# Autodesk Inventor assembly: ASY Мешалка
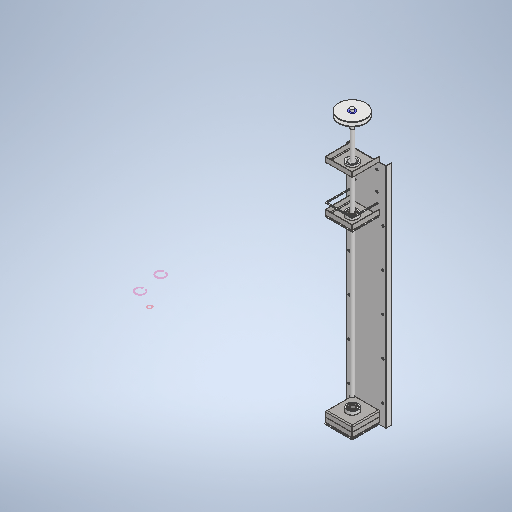
[picture p0: Inventor's stored thumbnail of the model, 512x512]
Saved by Autodesk Inventor 2025 (Build 290162010, 162A)
## iProperties
Created: 2024-04-09
Part Number: ASY Мешалка
Document SubType Name: Assembly
Designer: pokla
Author: pokla
## Documents named in this file (14)
- C:\Users\pokla\Documents\Inventor\Мешалка\ASY Мешалка.iam
- C:\Users\pokla\Documents\Inventor\Мешалка\SKF B7203 BE.ipt
- C:\Users\pokla\Documents\Inventor\Мешалка\Вал.ipt
- C:\Users\pokla\Documents\Inventor\Мешалка\дистанс.втулка.ipt
- C:\Users\pokla\Documents\Inventor\Мешалка\Втулка.ipt
- C:\Users\pokla\Documents\Inventor\Мешалка\CSN 02 9401 - G 17x40x7 - NBR.ipt
- C:\Users\pokla\Documents\Inventor\Мешалка\Шкив 119 мм.ipt
- Шкив 119 мм.ipt
- C:\Users\pokla\Documents\Inventor\Мешалка\Втулка для шкива.ipt
- C:\Users\pokla\Documents\Inventor\Content Center Files\R2024\en-US\ANSI B 27.7M(2)\ANSI B 27.7M - 3AMI-17.ipt
- C:\Users\pokla\Documents\Inventor\Content Center Files\R2024\en-US\ANSI B 27.7M(1)\ANSI B 27.7M - 3BMI-40.ipt
- C:\Users\pokla\Documents\Inventor\Мешалка\ASY Мешалка 2.0.iam
- C:\Users\pokla\Documents\Inventor\Мешалка\Седло для сальника.ipt
- C:\Users\pokla\Documents\Inventor\Мешалка\Седло для подшипника.ipt
## Components (17 placed, 12 different names)
1. Вал:1 — Mate:12, Insert:10, Mate:13, Insert:11
2. дистанс.втулка:1
3. SKF B- Angular contact SKF B7203 BE:2 — Rigid:5
4. SKF B- Angular contact SKF B7203 BE:3 — Rigid:4
5. Втулка:1 — Mate:12
6. CSN 02 9401 G G 17x40x7 - NBR:1 — Rotational:1
7. CSN 02 9401 G G 17x40x7 - NBR:2 — Rotational:2
8. Шкив 119 мм:1 — Insert:8, Mate:13
9. Втулка для шкива:1 — Insert:8, Insert:10
10. ANSI B 27.7M 3AMI-17:1
11. ANSI B 27.7M 3BMI-40:1
12. ANSI B 27.7M 3BMI-40:2
13. ASY Мешалка 2.0:1 [sub-assembly] — Rigid:2, Rigid:3, Rotational:3, Rotational:4, Flush:1, Flush:2, Flush:3
14. Седло для сальника:1 — Rigid:3, Rotational:1, Insert:11
15. Седло для сальника:2 — Rigid:2, Rotational:2
16. Седло для подшипника:1 — Rotational:3, Rigid:5
17. Седло для подшипника:2 — Rotational:4, Rigid:4
## Relationships (16: WeldJoint 4, RevoluteJoint 4, Insert 3, Flush 3, Mate 2)
- Insert:8: Шкив 119 мм:1 ↔ Втулка для шкива:1
- Mate:12: Вал:1 ↔ Втулка:1
- Insert:10 (10 mm): Вал:1 ↔ Втулка для шкива:1
- Mate:13: Вал:1 ↔ Шкив 119 мм:1
- Rigid:2 [WeldJoint]: ASY Мешалка 2.0:1 ↔ Седло для сальника:2
- Rigid:3 [WeldJoint]: ASY Мешалка 2.0:1 ↔ Седло для сальника:1
- Rotational:1 [RevoluteJoint]: CSN 02 9401 G G 17x40x7 - NBR:1 ↔ Седло для сальника:1
- Rotational:2 [RevoluteJoint]: CSN 02 9401 G G 17x40x7 - NBR:2 ↔ Седло для сальника:2
- Rotational:3 [RevoluteJoint]: ASY Мешалка 2.0:1 ↔ Седло для подшипника:1
- Rotational:4 [RevoluteJoint]: ASY Мешалка 2.0:1 ↔ Седло для подшипника:2
- Rigid:4 [WeldJoint]: SKF B- Angular contact SKF B7203 BE:3 ↔ Седло для подшипника:2
- Rigid:5 [WeldJoint]: SKF B- Angular contact SKF B7203 BE:2 ↔ Седло для подшипника:1
- Flush:1: ASY Мешалка 2.0:1
- Flush:2: ASY Мешалка 2.0:1
- Flush:3: ASY Мешалка 2.0:1
- Insert:11 (-200 mm): Вал:1 ↔ Седло для сальника:1
